# Autodesk Inventor assembly: leg
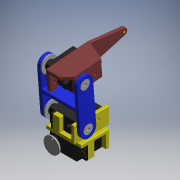
[picture p0: Inventor's stored thumbnail of the model, 180x180]
Saved by Autodesk Inventor 2017 (Build 210142000, 142)
## iProperties
Part Number: leg
Document SubType Name: Assembly
Designer: Alexander Miller
Author: Alexander Miller
## Documents named in this file (6)
- D:\Daten\Documents\Git\Hexapod\3DParts\leg.iam
- D:\Daten\Documents\Git\Hexapod\3DParts\Serov_with_arm.iam
- D:\Daten\Documents\Git\Hexapod\3DParts\Upper_leg.ipt
- D:\Daten\Documents\Git\Hexapod\3DParts\Middle_leg.ipt
- D:\Daten\Documents\Git\Hexapod\3DParts\Lower_leg.ipt
- D:\Daten\Documents\Git\Hexapod\3DParts\ball_bearing.ipt
## Components (10 placed, 5 different names)
1. Serov_with_arm:1 [sub-assembly] — Rotational:1, Rigid:13
2. Serov_with_arm:2 [sub-assembly] — Rigid:8
3. Upper_leg:1 — Rigid:13, Rigid:14
4. Upper_leg:2 — Rigid:8, Rigid:14
5. Middle_leg:1 — Rotational:1, Rigid:10, Rigid:12
6. Middle_leg:2 — Rigid:10, Rotational:2, Rigid:11
7. Serov_with_arm:3 [sub-assembly] — Rigid:9, Rotational:2
8. Lower_leg:1 — Rigid:9
9. ball_bearing:1 — Rigid:11
10. ball_bearing:2 — Rigid:12
## Relationships (9: WeldJoint 7, RevoluteJoint 2)
- Rotational:1 [RevoluteJoint]: Serov_with_arm:1 ↔ Middle_leg:1
- Rigid:8 [WeldJoint]: Serov_with_arm:2 ↔ Upper_leg:2
- Rigid:9 [WeldJoint]: Serov_with_arm:3 ↔ Lower_leg:1
- Rigid:10 [WeldJoint]: Middle_leg:1 ↔ Middle_leg:2
- Rotational:2 [RevoluteJoint]: Middle_leg:2 ↔ Serov_with_arm:3
- Rigid:11 [WeldJoint]: Middle_leg:2 ↔ ball_bearing:1
- Rigid:12 [WeldJoint]: Middle_leg:1 ↔ ball_bearing:2
- Rigid:13 [WeldJoint]: Serov_with_arm:1 ↔ Upper_leg:1
- Rigid:14 [WeldJoint]: Upper_leg:1 ↔ Upper_leg:2
